# Autodesk Inventor assembly: ShooterPrototype-ver1-1111-2019
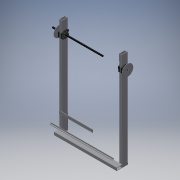
[picture p0: Inventor's stored thumbnail of the model, 180x180]
Saved by Autodesk Inventor 2018 (Build 220112000, 112)
## iProperties
Created: 2020-01-17
Part Number: ShooterPrototype-ver1-1111-2019
Document SubType Name: Assembly
Designer: JMHal
Author: JMHal
## Documents named in this file (9)
- E:\GrabCAD\Power Hawks CAD\2020 Infinite Recharge\Shooting\Assemblies\ShooterPrototype-ver1-1111-2019.iam
- E:\GrabCAD\Power Hawks CAD\2020 Infinite Recharge\Shooting\Parts\12in 2x1 Aluminum Block-ver1-1111-2019.ipt
- E:\GrabCAD\Power Hawks CAD\2020 Infinite Recharge\Shooting\Parts\16in 2x1 Aluminum Block-ver1-1111-2019.ipt
- E:\GrabCAD\Power Hawks CAD\2020 Infinite Recharge\Shooting\Parts\19 in L Block-ver1-1111-2019.ipt
- E:\GrabCAD\Power Hawks CAD\2020 Infinite Recharge\Shooting\Parts\12in Aluminum Plate-ver-1-1111-2019.ipt
- E:\GrabCAD\Power Hawks CAD\Resources\Chassis Parts\0.5inThunderHexShaft(18in)-1111-2016.ipt
- E:\GrabCAD\Power Hawks CAD\2020 Infinite Recharge\Shooting\Parts\VersaBlock-ver1-1111-2019.ipt
- E:\GrabCAD\Power Hawks CAD\Resources\VEXpro Resources\Bearings\0.5inHexFlangedBearing(1.125inx0.313in)-1111-2016.ipt
- E:\GrabCAD\Power Hawks CAD\2020 Infinite Recharge\Shooting\Parts\4in Wheel Plate-ver1-1111-2019.ipt
## Components (16 placed, 8 different names)
1. 12in 2x1 Aluminum Block-ver1-1111-2019:1 — Mate:4, Mate:5, Mate:6, Mate:7, Mate:8, Mate:9, Mate:10, Mate:11, Mate:14
2. 19 in L Block-ver1-1111-2019:1 — Mate:4, Mate:5
3. 12in Aluminum Plate-ver-1-1111-2019:1 — Mate:12, Mate:13, Mate:14
4. 16in 2x1 Aluminum Block-ver1-1111-2019:3 — Mate:6, Mate:7, Mate:8, Mate:12, Mate:13, Mate:15, Cylindrical:2, Mate:16, Angle:1, Cylindrical:5, Mate:18, Angle:3
5. 16in 2x1 Aluminum Block-ver1-1111-2019:4 — Mate:9, Mate:10, Mate:11, Cylindrical:3, Mate:17, Angle:2, Cylindrical:6, Mate:19, Angle:4, Mate:20
6. 0.5inThunderHexShaft(18in)-1111-2016:1 — Cylindrical:7, Cylindrical:8, Cylindrical:9
7. VersaBlock-ver1-1111-2019:1 — Mate:15, Angle:1, Rotational:1
8. 0.5inHexFlangedBearing(1.125inx0.313in)-1111-2016:1 — Cylindrical:2, Mate:16, Rotational:1, Cylindrical:7
9. 0.5inHexFlangedBearing(1.125inx0.313in)-1111-2016:2 — Cylindrical:3, Mate:17, Rotational:2
10. VersaBlock-ver1-1111-2019:2 — Rotational:2, Angle:2
11. 0.5inHexFlangedBearing(1.125inx0.313in)-1111-2016:3 — Cylindrical:5, Mate:18, Rotational:3
12. VersaBlock-ver1-1111-2019:3 — Rotational:3, Angle:3
13. VersaBlock-ver1-1111-2019:4 — Rotational:4, Angle:4
14. 0.5inHexFlangedBearing(1.125inx0.313in)-1111-2016:4 — Cylindrical:6, Mate:19, Rotational:4
15. 4in Wheel Plate-ver1-1111-2019:1 — Cylindrical:8
16. 4in Wheel Plate-ver1-1111-2019:2 — Cylindrical:9, Mate:20
## Relationships (32: Mate 17, CylindricalJoint 7, Angle 4, RevoluteJoint 4)
- Mate:4: 12in 2x1 Aluminum Block-ver1-1111-2019:1 ↔ 19 in L Block-ver1-1111-2019:1
- Mate:5: 12in 2x1 Aluminum Block-ver1-1111-2019:1 ↔ 19 in L Block-ver1-1111-2019:1
- Mate:6: 12in 2x1 Aluminum Block-ver1-1111-2019:1 ↔ 16in 2x1 Aluminum Block-ver1-1111-2019:3
- Mate:7: 12in 2x1 Aluminum Block-ver1-1111-2019:1 ↔ 16in 2x1 Aluminum Block-ver1-1111-2019:3
- Mate:8: 12in 2x1 Aluminum Block-ver1-1111-2019:1 ↔ 16in 2x1 Aluminum Block-ver1-1111-2019:3
- Mate:9: 12in 2x1 Aluminum Block-ver1-1111-2019:1 ↔ 16in 2x1 Aluminum Block-ver1-1111-2019:4
- Mate:10: 12in 2x1 Aluminum Block-ver1-1111-2019:1 ↔ 16in 2x1 Aluminum Block-ver1-1111-2019:4
- Mate:11: 12in 2x1 Aluminum Block-ver1-1111-2019:1 ↔ 16in 2x1 Aluminum Block-ver1-1111-2019:4
- Mate:12: 12in Aluminum Plate-ver-1-1111-2019:1 ↔ 16in 2x1 Aluminum Block-ver1-1111-2019:3
- Mate:13: 12in Aluminum Plate-ver-1-1111-2019:1 ↔ 16in 2x1 Aluminum Block-ver1-1111-2019:3
- Mate:14 (152.4 mm): 12in 2x1 Aluminum Block-ver1-1111-2019:1 ↔ 12in Aluminum Plate-ver-1-1111-2019:1
- Mate:15: 16in 2x1 Aluminum Block-ver1-1111-2019:3 ↔ VersaBlock-ver1-1111-2019:1
- Cylindrical:2: 16in 2x1 Aluminum Block-ver1-1111-2019:3 ↔ 0.5inHexFlangedBearing(1.125inx0.313in)-1111-2016:1
- Mate:16: 16in 2x1 Aluminum Block-ver1-1111-2019:3 ↔ 0.5inHexFlangedBearing(1.125inx0.313in)-1111-2016:1
- Cylindrical:3: 16in 2x1 Aluminum Block-ver1-1111-2019:4 ↔ 0.5inHexFlangedBearing(1.125inx0.313in)-1111-2016:2
- Mate:17: 16in 2x1 Aluminum Block-ver1-1111-2019:4 ↔ 0.5inHexFlangedBearing(1.125inx0.313in)-1111-2016:2
- Angle:1 (0 deg): 16in 2x1 Aluminum Block-ver1-1111-2019:3 ↔ VersaBlock-ver1-1111-2019:1
- Rotational:1 [RevoluteJoint]: VersaBlock-ver1-1111-2019:1 ↔ 0.5inHexFlangedBearing(1.125inx0.313in)-1111-2016:1
- Rotational:2 [RevoluteJoint]: 0.5inHexFlangedBearing(1.125inx0.313in)-1111-2016:2 ↔ VersaBlock-ver1-1111-2019:2
- Angle:2 (0 deg): 16in 2x1 Aluminum Block-ver1-1111-2019:4 ↔ VersaBlock-ver1-1111-2019:2
- Cylindrical:5: 16in 2x1 Aluminum Block-ver1-1111-2019:3 ↔ 0.5inHexFlangedBearing(1.125inx0.313in)-1111-2016:3
- Mate:18: 16in 2x1 Aluminum Block-ver1-1111-2019:3 ↔ 0.5inHexFlangedBearing(1.125inx0.313in)-1111-2016:3
- Rotational:3 [RevoluteJoint]: 0.5inHexFlangedBearing(1.125inx0.313in)-1111-2016:3 ↔ VersaBlock-ver1-1111-2019:3
- Angle:3 (0 deg): 16in 2x1 Aluminum Block-ver1-1111-2019:3 ↔ VersaBlock-ver1-1111-2019:3
- Cylindrical:6: 16in 2x1 Aluminum Block-ver1-1111-2019:4 ↔ 0.5inHexFlangedBearing(1.125inx0.313in)-1111-2016:4
- Mate:19: 16in 2x1 Aluminum Block-ver1-1111-2019:4 ↔ 0.5inHexFlangedBearing(1.125inx0.313in)-1111-2016:4
- Rotational:4 [RevoluteJoint]: VersaBlock-ver1-1111-2019:4 ↔ 0.5inHexFlangedBearing(1.125inx0.313in)-1111-2016:4
- Angle:4 (0 deg): 16in 2x1 Aluminum Block-ver1-1111-2019:4 ↔ VersaBlock-ver1-1111-2019:4
- Cylindrical:7: 0.5inThunderHexShaft(18in)-1111-2016:1 ↔ 0.5inHexFlangedBearing(1.125inx0.313in)-1111-2016:1
- Cylindrical:8: 0.5inThunderHexShaft(18in)-1111-2016:1 ↔ 4in Wheel Plate-ver1-1111-2019:1
- Cylindrical:9: 0.5inThunderHexShaft(18in)-1111-2016:1 ↔ 4in Wheel Plate-ver1-1111-2019:2
- Mate:20 (23.7998 mm): 16in 2x1 Aluminum Block-ver1-1111-2019:4 ↔ 4in Wheel Plate-ver1-1111-2019:2
